# Autodesk Inventor assembly: CAD Model of Bridge Assembly
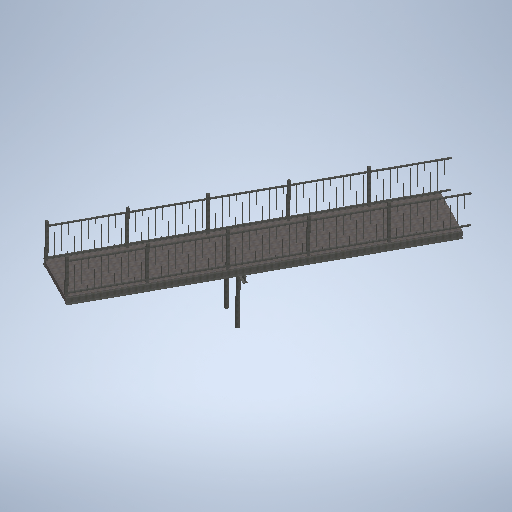
[picture p0: Inventor's stored thumbnail of the model, 512x512]
Saved by Autodesk Inventor 2025 (Build 290162000, 162)
## iProperties
Created: 2024-06-26
Part Number: CAD Model of Bridge Assembly
Document SubType Name: Assembly
Designer: track
Author: track
## Documents named in this file (7)
- C:\Users\track\OneDrive\Documents\USC-walking-bridges\Bridge_A\CAD_model\CAD Model of Bridge Assembly.iam
- C:\Users\track\OneDrive\Documents\USC-walking-bridges\Bridge_A\CAD_model\Concrete Walkway.ipt
- C:\Users\track\OneDrive\Documents\USC-walking-bridges\Bridge_A\CAD_model\Long I-Beam.ipt
- C:\Users\track\OneDrive\Documents\USC-walking-bridges\Bridge_A\CAD_model\Cylinder Supports.ipt
- C:\Users\track\OneDrive\Documents\USC-walking-bridges\Bridge_A\CAD_model\Short I-Beam.ipt
- C:\Users\track\OneDrive\Documents\USC-walking-bridges\Bridge_A\CAD_model\Railing.ipt
- C:\Users\track\OneDrive\Documents\USC-walking-bridges\Bridge_A\CAD_model\Cross Supports.ipt
## Components (16 placed, 6 different names)
1. Concrete Walkway:1 — Mate:1, Mate:2, Flush:2, Flush:3, Flush:4, Flush:6, Mate:18, Flush:7, Flush:8, Mate:19, Flush:9, Flush:10, Mate:21, Mate:22, Flush:11, Mate:23, Mate:24, Flush:12
2. Long I-Beam:1 — Flush:1, Mate:4, Flush:3, Flush:6, Mate:18, Flush:7, Flush:8
3. Cylinder Supports:1 — Mate:5, Slider:1, Mate:17
4. Short I-Beam:1 — Flush:1, Mate:4, Flush:2, Mate:5, Slider:1, Mate:17
5. Cross Supports:1 — Mate:1, Mate:2, Mate:20
6. Long I-Beam:2 — Flush:4, Mate:19, Flush:9, Flush:10, Mate:20
7. Railing:1 — Mate:21, Mate:22, Flush:11
8. Railing:3
9. Railing:4
10. Railing:5
11. Railing:6
12. Railing:2 — Mate:23, Mate:24, Flush:12
13. Railing:7
14. Railing:8
15. Railing:9
16. Railing:10
## Component patterns: (5 elements, first: Railing:1), (5 elements, first: Railing:2)
## Relationships (24: Mate 12, Flush 11, TranslationJoint 1)
- Mate:1 (381 mm): Concrete Walkway:1 ↔ Cross Supports:1
- Mate:2: Concrete Walkway:1 ↔ Cross Supports:1
- Flush:1 (-120.65 mm): Long I-Beam:1 ↔ Short I-Beam:1
- Mate:4: Long I-Beam:1 ↔ Short I-Beam:1
- Flush:2 (4375.15 mm): Concrete Walkway:1 ↔ Short I-Beam:1
- Mate:5: Cylinder Supports:1 ↔ Short I-Beam:1
- Flush:3: Concrete Walkway:1 ↔ Long I-Beam:1
- Flush:4: Concrete Walkway:1 ↔ Long I-Beam:2
- Flush:6: Concrete Walkway:1 ↔ Long I-Beam:1
- Slider:1 [TranslationJoint]: Cylinder Supports:1 ↔ Short I-Beam:1
- Mate:17 (-533.4 mm): Cylinder Supports:1 ↔ Short I-Beam:1
- Mate:18: Concrete Walkway:1 ↔ Long I-Beam:1
- Flush:7: Concrete Walkway:1 ↔ Long I-Beam:1
- Flush:8: Concrete Walkway:1 ↔ Long I-Beam:1
- Mate:19: Concrete Walkway:1 ↔ Long I-Beam:2
- Flush:9: Concrete Walkway:1 ↔ Long I-Beam:2
- Flush:10: Concrete Walkway:1 ↔ Long I-Beam:2
- Mate:20: Cross Supports:1 ↔ Long I-Beam:2
- Mate:21: Concrete Walkway:1 ↔ Railing:1
- Mate:22: Concrete Walkway:1 ↔ Railing:1
- Flush:11: Concrete Walkway:1 ↔ Railing:1
- Mate:23: Concrete Walkway:1 ↔ Railing:2
- Mate:24: Concrete Walkway:1 ↔ Railing:2
- Flush:12: Concrete Walkway:1 ↔ Railing:2
